# Autodesk Inventor assembly: Assembly2
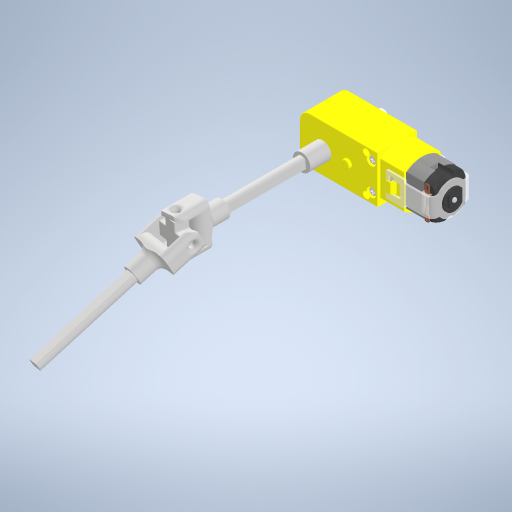
[picture p0: Inventor's stored thumbnail of the model, 512x512]
Saved by Autodesk Inventor 2023.2 (Build 272271000, 271)
## iProperties
Created: 2022-11-25
Part Number: Assembly2
Document SubType Name: Assembly
Designer: omrfrkmll
Author: omrfrkmll
## Documents named in this file (6)
- C:\Users\omr_f\Desktop\mechanism design project\Assembly2.iam
- C:\Users\omr_f\Desktop\mechanism design project\6v dc torque motor.iam
- C:\Users\omr_f\Desktop\mechanism design project\bağlantı elemanı.ipt
- C:\Users\omr_f\Desktop\mechanism design project\şaft.ipt
- C:\Users\omr_f\Desktop\mechanism design project\differantial.ipt
- C:\Users\omr_f\Desktop\mechanism design project\universal bağlantı.ipt
## Components (7 placed, 5 different names)
1. 6v dc torque motor:1 [sub-assembly] — Mate:1, Mate:2, Mate:3, Mate:6
2. bağlantı elemanı:1 — Mate:1, Flush:1, Mate:3, Mate:4
3. şaft:1 — Mate:4, Mate:5, Mate:6, Mate:7, Mate:8, Mate:11
4. differantial:1 — Mate:7, Mate:8, Mate:9, Mate:11, Mate:12
5. universal bağlantı:1 — Mate:9, Mate:12, Mate:13, Mate:14
6. differantial:2 — Mate:13, Mate:14, Mate:15, Mate:16, Mate:17
7. şaft:2 — Mate:15, Mate:16, Mate:17
## Relationships (17: Mate 16, Flush 1)
- Mate:1: 6v dc torque motor:1 ↔ bağlantı elemanı:1
- Flush:1 (0.05 mm): bağlantı elemanı:1
- Mate:2: 6v dc torque motor:1
- Mate:3: 6v dc torque motor:1 ↔ bağlantı elemanı:1
- Mate:4: bağlantı elemanı:1 ↔ şaft:1
- Mate:5: şaft:1
- Mate:6: 6v dc torque motor:1 ↔ şaft:1
- Mate:7: şaft:1 ↔ differantial:1
- Mate:8: şaft:1 ↔ differantial:1
- Mate:9: differantial:1 ↔ universal bağlantı:1
- Mate:11: şaft:1 ↔ differantial:1
- Mate:12: differantial:1 ↔ universal bağlantı:1
- Mate:13: universal bağlantı:1 ↔ differantial:2
- Mate:14: universal bağlantı:1 ↔ differantial:2
- Mate:15: differantial:2 ↔ şaft:2
- Mate:16: differantial:2 ↔ şaft:2
- Mate:17 (-5 mm): differantial:2 ↔ şaft:2
